# Autodesk Inventor assembly: G3D_Mech_Endstop
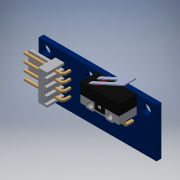
[picture p0: Inventor's stored thumbnail of the model, 180x180]
Saved by Autodesk Inventor 2016 SP1 (Build 200210100, 210)
## iProperties
Created: 2014-03-19
Part Number: G3D_Mech_Endstop
Document SubType Name: Assembly
Designer: iLyngklip
Sending System: SolidWorks 2014
Last Author: roberto
Last Saved: 2014-03-19
Author: iLyngklip
## Documents named in this file (4)
- C:\Users\PowerStation9000\AppData\Local\Autodesk\Autodesk Sync\Cloud\mathiaslk\UltiBot mk2\Importerede komponenter\Mech endstop\G3D_Mech_Endstop.iam
- C:\Users\PowerStation9000\AppData\Local\Autodesk\Autodesk Sync\Cloud\mathiaslk\UltiBot mk2\Importerede komponenter\Mech endstop\PCB_Mech_Endstop.ipt
- C:\Users\PowerStation9000\AppData\Local\Autodesk\Autodesk Sync\Cloud\mathiaslk\UltiBot mk2\Importerede komponenter\Mech endstop\Endstop.iam
- C:\Users\PowerStation9000\AppData\Local\Autodesk\Autodesk Sync\Cloud\mathiaslk\UltiBot mk2\Importerede komponenter\Mech endstop\SIL_4_P_90DEG.ipt
## Components (3 placed, 3 different names)
1. PCB_Mech_Endstop:1 — Flush:1, Flush:2, Flush:3, Flush:4
2. Endstop:1 [sub-assembly] — Flush:1, Flush:2
3. SIL_4_P_90DEG:1 — Flush:3, Flush:4
## Relationships (4: Flush 4)
- Flush:1: PCB_Mech_Endstop:1 ↔ Endstop:1
- Flush:2 (6.611 mm): PCB_Mech_Endstop:1 ↔ Endstop:1
- Flush:3 (3.05 mm): PCB_Mech_Endstop:1 ↔ SIL_4_P_90DEG:1
- Flush:4 (5.6 mm): PCB_Mech_Endstop:1 ↔ SIL_4_P_90DEG:1
